# Autodesk Inventor assembly: 606
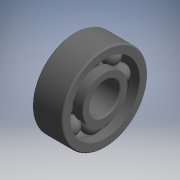
[picture p0: Inventor's stored thumbnail of the model, 180x180]
Saved by Autodesk Inventor 2017.3 (Build 213256000, 256)
## iProperties
Category: PARTsolutions
Company: NSK_RB
Part Number: 606
Catalog Web Link: www.cadenas.de
Description: Open Type-
Vendor: NSK_RB
Document SubType Name: Assembly
Designer: partserver
Manufacturer: NSK_RB
Mass: 0.771262 g
Surface Area: 13.6121 cm^2
Volume: 0.771262 cm^3
Density: 1 g/cm^3
Title: 606
Author: Cadenas PARTsolutions
PSOL_IDENT_0: {$CADENAS_DATA\23d-libs\nsk_rb\roller_bearings\deep_groove_bb\exstra_small_miniatur_bb\metric_design
PSOL_IDENT_1: \open_type_asmtab.prj},156 {VTYP=3D},{STYP=ASSTAB},{NB=606},{LINA=606},{NN=Open Type},{DATE=10.04.20
PSOL_IDENT_2: 20 04:57:45},{GEOMDATE=04.01.2008},{VERSION=},{LINEID=1680},{WBVAR=},{WBNUMERIC=}  {NB=606},{LINA=60
PSOL_IDENT_3: 6},{KT=DUMMY},{IDNR=},{STAN=Standard},{ORDER=606},{SD=6.0},{X=6.0},{DI1=8.92},{SDE1=13.75},{D=17},{D
PSOL_IDENT_4: D=17},{B=6.0},{B1=0.0},{R=0.30},{R1=0.00},{CR1=2260},{COR1=835},{CR2=231},{COR2=85.0},{LG=38000},{LO=
PSOL_IDENT_5: 45000},{DA=8.0},{DB=0.0},{DA1=15.0},{DB1=0.0},{RA=0.30},{RB=0.00},{MASS=5.97},{SC=1},{PPATH=open_typ
PSOL_IDENT_6: e_asmtpl.prj}
NB: 606
NN: Open Type
NBSYN: $ORDER.
LINA: 606
CATALOG: NSK Rolling Bearing
STAN: Standard
ORDER: 606
SD: 6
D: 17
B: 6
R: 0.3
CR1: 2260
COR1: 835
CR2: 231
COR2: 85
LG: 38000
LO: 45000
DA: 8
DA1: 15
RA: 0.3
MASS: 5.97
SUPPLIER: NSK_RB
ARTICLENO: 606
BOMINFO: 606
CREATOR: CADENAS GmbH
## Documents named in this file (4)
- e:\temp\worker_32\temp\exporttempdir_316_46_rY9NJ\format_0\606.iam
- e:\temp\worker_32\temp\exporttempdir_316_46_rY9NJ\format_0\606 Outer Ring.ipt
- e:\temp\worker_32\temp\exporttempdir_316_46_rY9NJ\format_0\606 Inner Ring.ipt
- e:\temp\worker_32\temp\exporttempdir_316_46_rY9NJ\format_0\606 Ball.ipt
## Components (10 placed, 3 different names)
1. 606 Outer Ring:1 — ip_ot_or_XY@1 <-> ip_op_ir_1a_XY@2, ip_ot_or_Z@1 <-> ip_op_ir_1a_Z@2, ip_ot_or_YZ@1 <-> ip_op_ir_1a_YZ@2
2. 606 Inner Ring:1 — ip_ot_or_XY@1 <-> ip_op_ir_1a_XY@2, ip_ot_or_Z@1 <-> ip_op_ir_1a_Z@2, ip_ot_or_YZ@1 <-> ip_op_ir_1a_YZ@2, ip_op_ir_1_1_XY@2 <-> ip_op_b_XY@3, ip_op_ir_1_1_Z@2 <-> ip_op_b_Z@3, ip_op_ir_1_1_YZ@2 <-> ip_op_b_YZ@3, ip_op_ir_1_2_XY@2 <-> ip_op_b_XY@4, ip_op_ir_1_2_Z@2 <-> ip_op_b_Z@4, ip_op_ir_1_2_YZ@2 <-> ip_op_b_YZ@4, ip_op_ir_1_3_XY@2 <-> ip_op_b_XY@5, ip_op_ir_1_3_Z@2 <-> ip_op_b_Z@5, ip_op_ir_1_3_YZ@2 <-> ip_op_b_YZ@5, ip_op_ir_1_4_XY@2 <-> ip_op_b_XY@6, ip_op_ir_1_4_Z@2 <-> ip_op_b_Z@6, ip_op_ir_1_4_YZ@2 <-> ip_op_b_YZ@6, ip_op_ir_1_5_XY@2 <-> ip_op_b_XY@7, ip_op_ir_1_5_Z@2 <-> ip_op_b_Z@7, ip_op_ir_1_5_YZ@2 <-> ip_op_b_YZ@7, ip_op_ir_1_6_XY@2 <-> ip_op_b_XY@8, ip_op_ir_1_6_Z@2 <-> ip_op_b_Z@8, ip_op_ir_1_6_YZ@2 <-> ip_op_b_YZ@8, ip_op_ir_1_7_XY@2 <-> ip_op_b_XY@9, ip_op_ir_1_7_Z@2 <-> ip_op_b_Z@9, ip_op_ir_1_7_YZ@2 <-> ip_op_b_YZ@9, ip_op_ir_1_8_XY@2 <-> ip_op_b_XY@10, ip_op_ir_1_8_Z@2 <-> ip_op_b_Z@10, ip_op_ir_1_8_YZ@2 <-> ip_op_b_YZ@10
3. 606 Ball:1 — ip_op_ir_1_1_XY@2 <-> ip_op_b_XY@3, ip_op_ir_1_1_Z@2 <-> ip_op_b_Z@3, ip_op_ir_1_1_YZ@2 <-> ip_op_b_YZ@3
4. 606 Ball:2 — ip_op_ir_1_2_XY@2 <-> ip_op_b_XY@4, ip_op_ir_1_2_Z@2 <-> ip_op_b_Z@4, ip_op_ir_1_2_YZ@2 <-> ip_op_b_YZ@4
5. 606 Ball:3 — ip_op_ir_1_3_XY@2 <-> ip_op_b_XY@5, ip_op_ir_1_3_Z@2 <-> ip_op_b_Z@5, ip_op_ir_1_3_YZ@2 <-> ip_op_b_YZ@5
6. 606 Ball:4 — ip_op_ir_1_4_XY@2 <-> ip_op_b_XY@6, ip_op_ir_1_4_Z@2 <-> ip_op_b_Z@6, ip_op_ir_1_4_YZ@2 <-> ip_op_b_YZ@6
7. 606 Ball:5 — ip_op_ir_1_5_XY@2 <-> ip_op_b_XY@7, ip_op_ir_1_5_Z@2 <-> ip_op_b_Z@7, ip_op_ir_1_5_YZ@2 <-> ip_op_b_YZ@7
8. 606 Ball:6 — ip_op_ir_1_6_XY@2 <-> ip_op_b_XY@8, ip_op_ir_1_6_Z@2 <-> ip_op_b_Z@8, ip_op_ir_1_6_YZ@2 <-> ip_op_b_YZ@8
9. 606 Ball:7 — ip_op_ir_1_7_XY@2 <-> ip_op_b_XY@9, ip_op_ir_1_7_Z@2 <-> ip_op_b_Z@9, ip_op_ir_1_7_YZ@2 <-> ip_op_b_YZ@9
10. 606 Ball:8 — ip_op_ir_1_8_XY@2 <-> ip_op_b_XY@10, ip_op_ir_1_8_Z@2 <-> ip_op_b_Z@10, ip_op_ir_1_8_YZ@2 <-> ip_op_b_YZ@10
## Relationships (27: Mate 17, Angle 9, Flush 1)
- ip_ot_or_XY@1 <-> ip_op_ir_1a_XY@2 [Flush]: 606 Outer Ring:1 ↔ 606 Inner Ring:1
- ip_ot_or_Z@1 <-> ip_op_ir_1a_Z@2 [Mate]: 606 Outer Ring:1 ↔ 606 Inner Ring:1
- ip_ot_or_YZ@1 <-> ip_op_ir_1a_YZ@2 [Angle] (90 deg): 606 Outer Ring:1 ↔ 606 Inner Ring:1
- ip_op_ir_1_1_XY@2 <-> ip_op_b_XY@3 [Mate]: 606 Inner Ring:1 ↔ 606 Ball:1
- ip_op_ir_1_1_Z@2 <-> ip_op_b_Z@3 [Mate]: 606 Inner Ring:1 ↔ 606 Ball:1
- ip_op_ir_1_1_YZ@2 <-> ip_op_b_YZ@3 [Angle] (0 deg): 606 Inner Ring:1 ↔ 606 Ball:1
- ip_op_ir_1_2_XY@2 <-> ip_op_b_XY@4 [Mate]: 606 Inner Ring:1 ↔ 606 Ball:2
- ip_op_ir_1_2_Z@2 <-> ip_op_b_Z@4 [Mate]: 606 Inner Ring:1 ↔ 606 Ball:2
- ip_op_ir_1_2_YZ@2 <-> ip_op_b_YZ@4 [Angle] (0 deg): 606 Inner Ring:1 ↔ 606 Ball:2
- ip_op_ir_1_3_XY@2 <-> ip_op_b_XY@5 [Mate]: 606 Inner Ring:1 ↔ 606 Ball:3
- ip_op_ir_1_3_Z@2 <-> ip_op_b_Z@5 [Mate]: 606 Inner Ring:1 ↔ 606 Ball:3
- ip_op_ir_1_3_YZ@2 <-> ip_op_b_YZ@5 [Angle] (0 deg): 606 Inner Ring:1 ↔ 606 Ball:3
- ip_op_ir_1_4_XY@2 <-> ip_op_b_XY@6 [Mate]: 606 Inner Ring:1 ↔ 606 Ball:4
- ip_op_ir_1_4_Z@2 <-> ip_op_b_Z@6 [Mate]: 606 Inner Ring:1 ↔ 606 Ball:4
- ip_op_ir_1_4_YZ@2 <-> ip_op_b_YZ@6 [Angle] (0 deg): 606 Inner Ring:1 ↔ 606 Ball:4
- ip_op_ir_1_5_XY@2 <-> ip_op_b_XY@7 [Mate]: 606 Inner Ring:1 ↔ 606 Ball:5
- ip_op_ir_1_5_Z@2 <-> ip_op_b_Z@7 [Mate]: 606 Inner Ring:1 ↔ 606 Ball:5
- ip_op_ir_1_5_YZ@2 <-> ip_op_b_YZ@7 [Angle] (0 deg): 606 Inner Ring:1 ↔ 606 Ball:5
- ip_op_ir_1_6_XY@2 <-> ip_op_b_XY@8 [Mate]: 606 Inner Ring:1 ↔ 606 Ball:6
- ip_op_ir_1_6_Z@2 <-> ip_op_b_Z@8 [Mate]: 606 Inner Ring:1 ↔ 606 Ball:6
- ip_op_ir_1_6_YZ@2 <-> ip_op_b_YZ@8 [Angle] (0 deg): 606 Inner Ring:1 ↔ 606 Ball:6
- ip_op_ir_1_7_XY@2 <-> ip_op_b_XY@9 [Mate]: 606 Inner Ring:1 ↔ 606 Ball:7
- ip_op_ir_1_7_Z@2 <-> ip_op_b_Z@9 [Mate]: 606 Inner Ring:1 ↔ 606 Ball:7
- ip_op_ir_1_7_YZ@2 <-> ip_op_b_YZ@9 [Angle] (0 deg): 606 Inner Ring:1 ↔ 606 Ball:7
- ip_op_ir_1_8_XY@2 <-> ip_op_b_XY@10 [Mate]: 606 Inner Ring:1 ↔ 606 Ball:8
- ip_op_ir_1_8_Z@2 <-> ip_op_b_Z@10 [Mate]: 606 Inner Ring:1 ↔ 606 Ball:8
- ip_op_ir_1_8_YZ@2 <-> ip_op_b_YZ@10 [Angle] (0 deg): 606 Inner Ring:1 ↔ 606 Ball:8
